# Autodesk Inventor assembly: poleStand
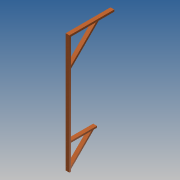
[picture p0: Inventor's stored thumbnail of the model, 180x180]
Saved by Autodesk Inventor 2014 SP1 (Build 180222100, 222)
## iProperties
Created: 2013-12-02
Part Number: poleStand
Document SubType Name: Assembly
Designer: Dave
Author: Dave
## Documents named in this file (6)
- C:\Users\Dave\Desktop\hera-cad\support\poleStandVertAssy.iam
- C:\Users\Dave\Desktop\hera-cad\support\poleStandVert.ipt
- C:\Users\Dave\Desktop\hera-cad\support\poleStandHoriz1.ipt
- C:\Users\Dave\Desktop\hera-cad\support\poleStand45.ipt
- C:\Users\Dave\Desktop\hera-cad\support\poleScreenHldHoriz.ipt
- C:\Users\Dave\Desktop\hera-cad\support\poleScreenHld45.ipt
## Components (5 placed, 5 different names)
1. poleStandVert:1 — Insert:1, Flush:3, Mate:1, Flush:4, Flush:5, Mate:3
2. poleStand45:1 — Insert:2, Flush:2, Flush:3
3. poleStandHoriz1:1 — Insert:1, Insert:2, Flush:2
4. poleScreenHldHoriz:1 — Mate:1, Flush:4, Flush:5, Mate:2, Flush:6
5. poleScreenHld45:1 — Mate:2, Mate:3, Flush:6
## Relationships (10: Flush 5, Mate 3, Insert 2)
- Insert:1: poleStandVert:1 ↔ poleStandHoriz1:1
- Insert:2: poleStand45:1 ↔ poleStandHoriz1:1
- Flush:2: poleStand45:1 ↔ poleStandHoriz1:1
- Flush:3: poleStandVert:1 ↔ poleStand45:1
- Mate:1: poleStandVert:1 ↔ poleScreenHldHoriz:1
- Flush:4: poleStandVert:1 ↔ poleScreenHldHoriz:1
- Flush:5: poleStandVert:1 ↔ poleScreenHldHoriz:1
- Mate:2: poleScreenHldHoriz:1 ↔ poleScreenHld45:1
- Mate:3: poleStandVert:1 ↔ poleScreenHld45:1
- Flush:6 (-1.651 mm): poleScreenHldHoriz:1 ↔ poleScreenHld45:1
